# Autodesk Inventor assembly: Poste de Travail - Quetzal
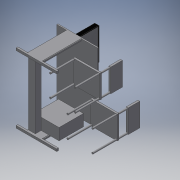
[picture p0: Inventor's stored thumbnail of the model, 180x180]
Saved by Autodesk Inventor 2016 SP1 (Build 200210100, 210)
## iProperties
Created: 2016-10-06
Part Number: Poste de Travail - Quetzal
Material: Générique
Document SubType Name: Assembly
Designer: dimercur
Author: dimercur
## Documents named in this file (4)
- D:\Users\dimercur\Documents\SVN\projets-gei\Salle 22-24\Poste de Travail - Quetzal.iam
- D:\Users\dimercur\Documents\SVN\projets-gei\Salle 22-24\Bureau-Quetzal-FormatPlus.ipt
- D:\Users\dimercur\Documents\SVN\projets-gei\Salle 22-24\Chaise.ipt
- D:\Users\dimercur\Documents\SVN\projets-gei\Salle 22-24\Ecran.ipt
## Components (4 placed, 3 different names)
1. Bureau-Quetzal-FormatPlus:1 — Affleurement:1, Affleurement:2, Placage:1, Placage:2, Placage:3, Placage:4, Placage:5, Placage:6, Placage:7
2. Chaise:1 — Affleurement:2, Placage:2, Placage:4
3. Chaise:2 — Affleurement:1, Placage:1, Placage:3
4. Ecran:1 — Placage:5, Placage:6, Placage:7
## Relationships (9: Mate 7, Flush 2)
- Affleurement:1 [Flush]: Bureau-Quetzal-FormatPlus:1 ↔ Chaise:2
- Affleurement:2 [Flush]: Bureau-Quetzal-FormatPlus:1 ↔ Chaise:1
- Placage:1 [Mate] (30 mm): Bureau-Quetzal-FormatPlus:1 ↔ Chaise:2
- Placage:2 [Mate] (30 mm): Bureau-Quetzal-FormatPlus:1 ↔ Chaise:1
- Placage:3 [Mate] (300 mm): Bureau-Quetzal-FormatPlus:1 ↔ Chaise:2
- Placage:4 [Mate] (600 mm): Bureau-Quetzal-FormatPlus:1 ↔ Chaise:1
- Placage:5 [Mate]: Bureau-Quetzal-FormatPlus:1 ↔ Ecran:1
- Placage:6 [Mate] (100 mm): Bureau-Quetzal-FormatPlus:1 ↔ Ecran:1
- Placage:7 [Mate] (300 mm): Bureau-Quetzal-FormatPlus:1 ↔ Ecran:1
